# Autodesk Inventor assembly: GP3-100
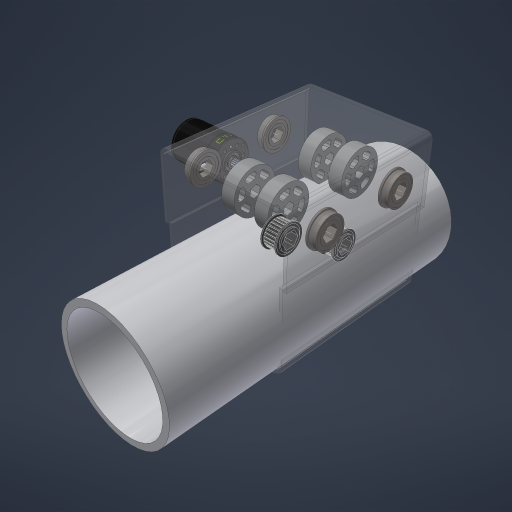
[picture p0: Inventor's stored thumbnail of the model, 512x512]
Saved by Autodesk Inventor 2023.4 (Build 274418000, 418)
## iProperties
Created: 2025-01-14
Part Number: GP3-100
Document SubType Name: Assembly
Designer: brand
Author: brand
## Documents named in this file (8)
- C:\Users\brand\OneDrive\Documents\GitHub\robotics 23\2025-ReefScape---CAD\Gripper\GP3\GP3-100.iam
- C:\Users\brand\OneDrive\Documents\GitHub\robotics 23\2025-ReefScape---CAD\Gripper\GP3\GP3-001.ipt
- C:\Users\brand\OneDrive\Documents\GitHub\robotics 23\2025-ReefScape---CAD\Gripper\GP3\GP3-002.ipt
- C:\Users\brand\OneDrive\Documents\GitHub\robotics 23\2025-ReefScape---CAD\Field Items\Game Pieces\GE-25500.ipt
- C:\Users\brand\OneDrive\Documents\GitHub\robotics 23\2025-ReefScape---CAD\COMMON PARTS\BEARINGS\0_500_Hex_ID_x_1_125_OD_x_0_313_WD_Flanged_Bearing_v2_217-3875.ipt
- C:\Users\brand\OneDrive\Documents\GitHub\robotics 23\2025-ReefScape---CAD\COMMON PARTS\WHEELS\1_625_OD_Straight_Flex_Wheel_217-6350.ipt
- C:\Users\brand\OneDrive\Documents\GitHub\robotics 23\2025-ReefScape---CAD\COMMON PARTS\MOTORS\Minion.ipt
- C:\Users\brand\OneDrive\Documents\GitHub\robotics 23\2025-ReefScape---CAD\COMMON PARTS\PULLEYS\gt2\24t_x_9mm_Wide_Double_Flange_Aluminum_Pulley_GT2_3mm_1_2_Hex_Bore_217-5875.ipt
## Components (14 placed, 7 different names)
1. GP3-001:1 — Angle:1, Flush:1, Mate:1, Insert:1, Insert:2, Insert:3, Insert:4, Mate:4
2. GP3-002:1 — Angle:1, Flush:1, Mate:1
3. GE-25500:1
4. 0_500_Hex_ID_x_1_125_OD_x_0_313_WD_Flanged_Bearing_v2_217-3875:1 — Insert:1
5. 0_500_Hex_ID_x_1_125_OD_x_0_313_WD_Flanged_Bearing_v2_217-3875:2 — Insert:2
6. 0_500_Hex_ID_x_1_125_OD_x_0_313_WD_Flanged_Bearing_v2_217-3875:3 — Insert:3, Mate:3
7. 0_500_Hex_ID_x_1_125_OD_x_0_313_WD_Flanged_Bearing_v2_217-3875:4 — Insert:4, Mate:2
8. 1_625_OD_Straight_Flex_Wheel_217-6350:1 — Mate:2
9. 1_625_OD_Straight_Flex_Wheel_217-6350:2 — Mate:3
10. 1_625_OD_Straight_Flex_Wheel_217-6350:3
11. 1_625_OD_Straight_Flex_Wheel_217-6350:4
12. Minion:1 — Mate:4
13. 24t_x_9mm_Wide_Double_Flange_Aluminum_Pulley_GT2_3mm_1_2_Hex_Bore_217-5875:1
14. 24t_x_9mm_Wide_Double_Flange_Aluminum_Pulley_GT2_3mm_1_2_Hex_Bore_217-5875:2
## Relationships (10: Mate 4, Insert 4, Angle 1, Flush 1)
- Angle:1 (0 deg): GP3-001:1 ↔ GP3-002:1
- Flush:1: GP3-001:1 ↔ GP3-002:1
- Mate:1: GP3-001:1 ↔ GP3-002:1
- Insert:1: GP3-001:1 ↔ 0_500_Hex_ID_x_1_125_OD_x_0_313_WD_Flanged_Bearing_v2_217-3875:1
- Insert:2: GP3-001:1 ↔ 0_500_Hex_ID_x_1_125_OD_x_0_313_WD_Flanged_Bearing_v2_217-3875:2
- Insert:3: GP3-001:1 ↔ 0_500_Hex_ID_x_1_125_OD_x_0_313_WD_Flanged_Bearing_v2_217-3875:3
- Insert:4: GP3-001:1 ↔ 0_500_Hex_ID_x_1_125_OD_x_0_313_WD_Flanged_Bearing_v2_217-3875:4
- Mate:2: 0_500_Hex_ID_x_1_125_OD_x_0_313_WD_Flanged_Bearing_v2_217-3875:4 ↔ 1_625_OD_Straight_Flex_Wheel_217-6350:1
- Mate:3: 0_500_Hex_ID_x_1_125_OD_x_0_313_WD_Flanged_Bearing_v2_217-3875:3 ↔ 1_625_OD_Straight_Flex_Wheel_217-6350:2
- Mate:4: GP3-001:1 ↔ Minion:1
